# Autodesk Inventor assembly: ЖестьСборка
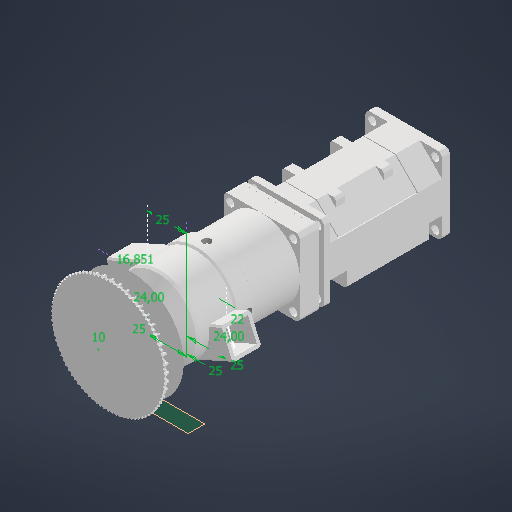
[picture p0: Inventor's stored thumbnail of the model, 512x512]
Saved by Autodesk Inventor 2026 (Build 300175000, 175)
## iProperties
Created: 2025-08-20
Part Number: ЖестьСборка
Document SubType Name: Assembly
Designer: seraf
Author: seraf
## Documents named in this file (10)
- E:\Документы\Github-rep\MIK-nozzle\Inventor модели\ЖестьСборка.iam
- E:\Документы\Github-rep\MIK-nozzle\Inventor модели\Корпус и двигатель\КорпДвиг.ipt
- E:\Документы\Github-rep\MIK-nozzle\Inventor модели\Корпус и двигатель\КрашкаКорпДвиг.ipt
- E:\Документы\Github-rep\MIK-nozzle\Inventor модели\Корпус и двигатель\Двигатель 3115.ipt
- E:\Документы\Github-rep\MIK-nozzle\Inventor модели\Корпус и двигатель\ПроставкаДвиг.ipt
- E:\Документы\Github-rep\MIK-nozzle\Inventor модели\Корпус и двигатель\КорпусЕСК.ipt
- E:\Документы\Github-rep\MIK-nozzle\Inventor модели\Корпус и двигатель\КрышкаЕСК.ipt
- E:\Документы\Github-rep\MIK-nozzle\Inventor модели\Ванна и диск\корпус ванночки.ipt
- E:\Документы\Github-rep\MIK-nozzle\Inventor модели\Ванна и диск\Статор без зубьев.ipt
- E:\Документы\Github-rep\MIK-nozzle\Inventor модели\Ванна и диск\Диск v2.ipt
## Components (9 placed, 9 different names)
1. КорпДвиг:1 — Совмещение:3, Совмещение:4, С поворотом:1, С поворотом:3
2. КрашкаКорпДвиг:1 — Жесткий:1, Совмещение:1, Совмещение:3, Совмещение:4
3. Двигатель 3115:1 — Совмещение:2
4. ПроставкаДвиг:1 — Жесткий:1, Совмещение:1, Совмещение:2
5. КорпусЕСК:1 — Заподлицо:1
6. КрышкаЕСК:1 — Заподлицо:1
7. корпус ванночки:1 — С поворотом:1, С поворотом:2
8. Статор без зубьев:1 — С поворотом:2
9. Диск v2:1 — С поворотом:3
## Relationships (9: Mate 4, RevoluteJoint 3, WeldJoint 1, Flush 1)
- Жесткий:1 [WeldJoint]: КрашкаКорпДвиг:1 ↔ ПроставкаДвиг:1
- Совмещение:1 [Mate]: КрашкаКорпДвиг:1 ↔ ПроставкаДвиг:1
- Совмещение:2 [Mate]: Двигатель 3115:1 ↔ ПроставкаДвиг:1
- Совмещение:3 [Mate]: КорпДвиг:1 ↔ КрашкаКорпДвиг:1
- Совмещение:4 [Mate]: КорпДвиг:1 ↔ КрашкаКорпДвиг:1
- Заподлицо:1 [Flush]: КорпусЕСК:1 ↔ КрышкаЕСК:1
- С поворотом:1 [RevoluteJoint]: КорпДвиг:1 ↔ корпус ванночки:1
- С поворотом:2 [RevoluteJoint]: корпус ванночки:1 ↔ Статор без зубьев:1
- С поворотом:3 [RevoluteJoint]: КорпДвиг:1 ↔ Диск v2:1
## Named parameters: Finish1_Area = 46.9357
note: some values were not read from the file. Shown as the stored number, unit unknown: "Finish1_Area".
